# Autodesk Inventor assembly: PULLEY ASSEMBLY
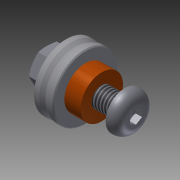
[picture p0: Inventor's stored thumbnail of the model, 180x180]
Saved by Autodesk Inventor 2013 (Build 170138000, 138)
## iProperties
Created: 2014-06-23
Part Number: PULLEY ASSEMBLY
Document SubType Name: Assembly
Designer: employee
Author: employee
## Documents named in this file (5)
- C:\Users\employee\Desktop\ConceptFORGE\ConceptFORGE\CoreXZ\PULLEY ASSEMBLY.iam
- C:\Users\employee\Desktop\ConceptFORGE\ConceptFORGE\CoreXZ\625vv.ipt
- C:\Users\employee\Desktop\ConceptFORGE\ConceptFORGE\CoreXZ\M5 NUT.ipt
- C:\Users\employee\Desktop\ConceptFORGE\ConceptFORGE\CoreXZ\M5X20.ipt
- C:\Users\employee\Desktop\ConceptFORGE\ConceptFORGE\CoreXZ\PULLEY SPACER.ipt
## Components (4 placed, 4 different names)
1. 625vv:1 — Insert:2, Insert:3
2. M5 NUT:1 — Insert:3
3. M5X20:1 — Insert:1
4. PULLEY SPACER:1 — Insert:1, Insert:2
## Relationships (3: Insert 3)
- Insert:1 (5.715 mm): M5X20:1 ↔ PULLEY SPACER:1
- Insert:2: 625vv:1 ↔ PULLEY SPACER:1
- Insert:3: 625vv:1 ↔ M5 NUT:1
